# Autodesk Inventor assembly: Quick Release Assy
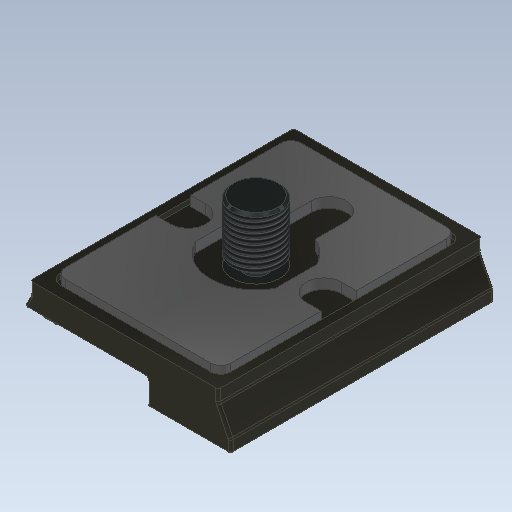
[picture p0: Inventor's stored thumbnail of the model, 512x512]
Saved by Autodesk Inventor 2020 (Build 240168000, 168)
## iProperties
Created: 2012-10-13
Part Number: Quick Release Assy
Document SubType Name: Assembly
Designer: Lance
Mass: 101.673 g
Surface Area: 107.817 cm^2
Volume: 15.0048 cm^3
Density: 6.77602 g/cm^3
Author: Lance
## Documents named in this file (4)
- C:\Users\Hesekiel\Desktop\MUM\Mechanika\Mechanizm elewacji i elektronika Filip\CAD\manfrotto-494rc2-tripod-head.snapshot.1\Manfrotto 494RC2 - Tripod Head\Quick Release Assy.iam
- C:\Users\Hesekiel\Desktop\MUM\Mechanika\Mechanizm elewacji i elektronika Filip\CAD\manfrotto-494rc2-tripod-head.snapshot.1\Manfrotto 494RC2 - Tripod Head\Quick Release Mounting.ipt
- C:\Users\Hesekiel\Desktop\MUM\Mechanika\Mechanizm elewacji i elektronika Filip\CAD\manfrotto-494rc2-tripod-head.snapshot.1\Manfrotto 494RC2 - Tripod Head\Thumb Screw Assy.iam
- C:\Users\Hesekiel\Desktop\MUM\Mechanika\Mechanizm elewacji i elektronika Filip\CAD\manfrotto-494rc2-tripod-head.snapshot.1\Manfrotto 494RC2 - Tripod Head\Quick Release Rubber Pad.ipt
## Components (3 placed, 3 different names)
1. Quick Release Mounting:1 — Insert:1, Angle:1, Mate:3, Mate:4, Angle:2
2. Thumb Screw Assy:1 [sub-assembly] — Insert:1, Angle:1
3. Quick Release Rubber Pad:1 — Mate:3, Mate:4, Angle:2
## Relationships (5: Angle 2, Mate 2, Insert 1)
- Insert:1: Quick Release Mounting:1 ↔ Thumb Screw Assy:1
- Angle:1 (180 deg): Quick Release Mounting:1 ↔ Thumb Screw Assy:1
- Mate:3: Quick Release Mounting:1 ↔ Quick Release Rubber Pad:1
- Mate:4: Quick Release Mounting:1 ↔ Quick Release Rubber Pad:1
- Angle:2 (180 deg): Quick Release Mounting:1 ↔ Quick Release Rubber Pad:1
